# Autodesk Inventor assembly: Assembly_Cube_Mirror_30x30_v3
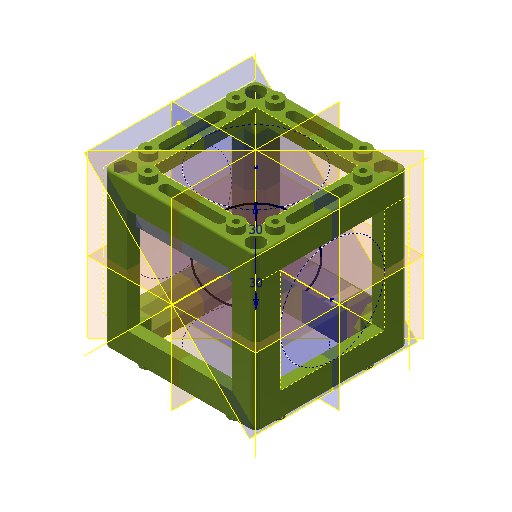
[picture p0: Inventor's stored thumbnail of the model, 512x512]
Saved by Autodesk Inventor 2022 (Build 260153000, 153)
## iProperties
Created: 2020-11-11
Part Number: Assembly_Cube_Mirror_30x30_v3
Document SubType Name: Assembly
Designer: marsikovabarbora
Author: marsikovabarbora
## Documents named in this file (4)
- C:\Users\PrakashLab\Documents\UC2-INVENTOR-Git\uc2_v3\Assembly_Cube_Mirror_30x30_v3.iam
- C:\Users\PrakashLab\Documents\UC2-INVENTOR-Git\uc2_v3\Assembly_Cube_empty_IM_v3.iam
- C:\Users\PrakashLab\Documents\UC2-INVENTOR-Git\uc2_v3\20_Cube_Insert_Mirror_Holder_wLogo_v3.ipt
- C:\Users\PrakashLab\Documents\UC2-INVENTOR-Git\uc2_v3\00_Mirror_30x30.ipt
## Components (3 placed, 3 different names)
1. Assembly_Cube_empty_IM_v3:1 [sub-assembly] — Mate:1, Mate:2, Mate:3, Mate:7, Mate:8, Mate:9
2. 20_Cube_Insert_Mirror_Holder_wLogo_v3:1 — Mate:5, Flush:2, Mate:6, Mate:7, Mate:8, Mate:9
3. 00_Mirror_30x30:1 — Mate:5, Flush:2, Mate:6
## Relationships (9: Mate 8, Flush 1)
- Mate:1: Assembly_Cube_empty_IM_v3:1
- Mate:2: Assembly_Cube_empty_IM_v3:1
- Mate:3: Assembly_Cube_empty_IM_v3:1
- Mate:5: 20_Cube_Insert_Mirror_Holder_wLogo_v3:1 ↔ 00_Mirror_30x30:1
- Flush:2: 20_Cube_Insert_Mirror_Holder_wLogo_v3:1 ↔ 00_Mirror_30x30:1
- Mate:6: 20_Cube_Insert_Mirror_Holder_wLogo_v3:1 ↔ 00_Mirror_30x30:1
- Mate:7: Assembly_Cube_empty_IM_v3:1 ↔ 20_Cube_Insert_Mirror_Holder_wLogo_v3:1
- Mate:8 (2 mm): Assembly_Cube_empty_IM_v3:1 ↔ 20_Cube_Insert_Mirror_Holder_wLogo_v3:1
- Mate:9: Assembly_Cube_empty_IM_v3:1 ↔ 20_Cube_Insert_Mirror_Holder_wLogo_v3:1
